# Autodesk Inventor assembly: Channel+Roller
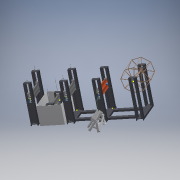
[picture p0: Inventor's stored thumbnail of the model, 180x180]
Saved by Autodesk Inventor 2019 (Build 230136000, 136)
## iProperties
Created: 2019-05-29
Part Number: Channel+Roller
Document SubType Name: Assembly
Designer: Satwik Pandey
Author: Satwik Pandey
## Documents named in this file (92)
- C:\Users\Satwik Pandey\Desktop\RuTAG Project\New folder\Channel+Roller.iam
- C:\Users\Satwik Pandey\Desktop\RuTAG Project\New folder\Channel1.ipt
- C:\Users\Satwik Pandey\Desktop\RuTAG Project\New folder\Channel2.ipt
- C:\Users\Satwik Pandey\Desktop\RuTAG Project\New folder\Extension.ipt
- C:\Users\Satwik Pandey\Desktop\RuTAG Project\New folder\Pillow Bearing inventor.ipt
- C:\Users\Satwik Pandey\Desktop\RuTAG Project\New folder\project rolller 1 part.ipt
- C:\Users\Satwik Pandey\Desktop\RuTAG Project\New folder\project rolller 1 part2.ipt
- C:\Users\Satwik Pandey\Desktop\RuTAG Project\New folder\project handle part(1).ipt
- C:\Users\Satwik Pandey\Desktop\RuTAG Project\New folder\Channel1_MIR.ipt
- C:\Users\Satwik Pandey\Desktop\RuTAG Project\New folder\Extension_MIR.ipt
- C:\Users\Satwik Pandey\Desktop\RuTAG Project\New folder\Pillow Bearing inventor_MIR.ipt
- C:\Users\Satwik Pandey\Desktop\RuTAG Project\New folder\Channel2_MIR.ipt
- C:\Users\Satwik Pandey\Desktop\RuTAG Project\New folder\project rolller 1 part_CPY.ipt
- C:\Users\Satwik Pandey\Desktop\RuTAG Project\New folder\project handle part(1)_CPY.ipt
- C:\Users\Satwik Pandey\Desktop\RuTAG Project\New folder\Channel1_MIR1.ipt
- C:\Users\Satwik Pandey\Desktop\RuTAG Project\New folder\Extension_MIR1.ipt
- C:\Users\Satwik Pandey\Desktop\RuTAG Project\New folder\Pillow Bearing inventor_MIR1.ipt
- C:\Users\Satwik Pandey\Desktop\RuTAG Project\New folder\Channel2_MIR1.ipt
- C:\Users\Satwik Pandey\Desktop\RuTAG Project\New folder\Channel1_MIR_MIR.ipt
- C:\Users\Satwik Pandey\Desktop\RuTAG Project\New folder\Extension_MIR_MIR.ipt
- C:\Users\Satwik Pandey\Desktop\RuTAG Project\New folder\Pillow Bearing inventor_MIR_MIR.ipt
- C:\Users\Satwik Pandey\Desktop\RuTAG Project\New folder\Channel2_MIR_MIR.ipt
- C:\Users\Satwik Pandey\Desktop\RuTAG Project\New folder\project handle part(1)_MIR1.ipt
- C:\Users\Satwik Pandey\Desktop\RuTAG Project\New folder\project roller 2 part1.ipt
- C:\Users\Satwik Pandey\Desktop\RuTAG Project\New folder\project roller 2 part 2.ipt
- C:\Users\Satwik Pandey\Desktop\RuTAG Project\New folder\steam pipe.ipt
- C:\Users\Satwik Pandey\Desktop\RuTAG Project\New folder\Rubber pipe.ipt
- C:\Users\Satwik Pandey\Desktop\RuTAG Project\New folder\solar heater 2.ipt
- C:\Users\Satwik Pandey\Desktop\RuTAG Project\New folder\RuTAG Roller_MIR.ipt
- C:\Users\Satwik Pandey\Desktop\RuTAG Project\New folder\Channel1_MIR4.ipt
- C:\Users\Satwik Pandey\Desktop\RuTAG Project\New folder\project flange bearing part1_MIR6.ipt
- C:\Users\Satwik Pandey\Desktop\RuTAG Project\New folder\project flange bearing part2_MIR5.ipt
- C:\Users\Satwik Pandey\Desktop\RuTAG Project\New folder\Channel1_MIR3_MIR.ipt
- C:\Users\Satwik Pandey\Desktop\RuTAG Project\New folder\project flange bearing part1_MIR5_MIR.ipt
- C:\Users\Satwik Pandey\Desktop\RuTAG Project\New folder\project flange bearing part2_MIR4_MIR.ipt
- C:\Users\Satwik Pandey\Desktop\RuTAG Project\New folder\Base1.ipt
- C:\Users\Satwik Pandey\Desktop\RuTAG Project\New folder\Base1_MIR.ipt
- C:\Users\Satwik Pandey\Desktop\RuTAG Project\New folder\Base2.ipt
- C:\Users\Satwik Pandey\Desktop\RuTAG Project\New folder\Base3.ipt
- C:\Users\Satwik Pandey\Desktop\RuTAG Project\New folder\Base4.ipt
- C:\Users\Satwik Pandey\Desktop\RuTAG Project\New folder\Channel1_MIR5.ipt
- C:\Users\Satwik Pandey\Desktop\RuTAG Project\New folder\Channel1_MIR_MIR2.ipt
- C:\Users\Satwik Pandey\Desktop\RuTAG Project\New folder\Channel1_MIR1_MIR.ipt
- C:\Users\Satwik Pandey\Desktop\RuTAG Project\New folder\Channel1_MIR_MIR_MIR.ipt
- C:\Users\Satwik Pandey\Desktop\RuTAG Project\New folder\LeadScrewArrangement.iam
- C:\Users\Satwik Pandey\Desktop\RuTAG Project\New folder\Cap1.ipt
- C:\Users\Satwik Pandey\Desktop\RuTAG Project\New folder\project handle part(1)_MIR1_MIR.ipt
- C:\Users\Satwik Pandey\Desktop\RuTAG Project\New folder\project roller 2 part1_MIR.ipt
- C:\Users\Satwik Pandey\Desktop\RuTAG Project\New folder\project roller 2 part 2_MIR.ipt
- C:\Users\Satwik Pandey\Desktop\RuTAG Project\New folder\Rubber pipe - Cap.ipt
- C:\Users\Satwik Pandey\Desktop\RuTAG Project\New folder\project flange bearing part2.ipt
- C:\Users\Satwik Pandey\Desktop\RuTAG Project\New folder\project flange bearing part1_MIR7.ipt
- C:\Users\Satwik Pandey\Desktop\RuTAG Project\New folder\project flange bearing part2_MIR6.ipt
- C:\Users\Satwik Pandey\Desktop\RuTAG Project\New folder\project flange bearing part1_MIR7_MIR.ipt
- C:\Users\Satwik Pandey\Desktop\RuTAG Project\New folder\Rubber pipe2.ipt
- C:\Users\Satwik Pandey\Desktop\RuTAG Project\New folder\Rubber pipe turn.ipt
- C:\Users\Satwik Pandey\Desktop\RuTAG Project\New folder\project flange bearing part2_MIR5_MIR.ipt
- C:\Users\Satwik Pandey\Desktop\RuTAG Project\New folder\Paste Container.ipt
- C:\Users\Satwik Pandey\Desktop\RuTAG Project\New folder\Extension_MIR3.ipt
- C:\Users\Satwik Pandey\Desktop\RuTAG Project\New folder\Pillow Bearing inventor_MIR3.ipt
- C:\Users\Satwik Pandey\Desktop\RuTAG Project\New folder\Channel2_MIR3.ipt
- C:\Users\Satwik Pandey\Desktop\RuTAG Project\New folder\Channel1_MIR6.ipt
- C:\Users\Satwik Pandey\Desktop\RuTAG Project\New folder\project rolller 1 part_MIR.ipt
- C:\Users\Satwik Pandey\Desktop\RuTAG Project\New folder\project handle part(1)_MIR2.ipt
- C:\Users\Satwik Pandey\Desktop\RuTAG Project\New folder\Extension_MIR_MIR2.ipt
- C:\Users\Satwik Pandey\Desktop\RuTAG Project\New folder\Pillow Bearing inventor_MIR_MIR2.ipt
- C:\Users\Satwik Pandey\Desktop\RuTAG Project\New folder\Channel2_MIR_MIR2.ipt
- C:\Users\Satwik Pandey\Desktop\RuTAG Project\New folder\Channel1_MIR_MIR3.ipt
- C:\Users\Satwik Pandey\Desktop\RuTAG Project\New folder\project rolller 1 part_CPY_MIR.ipt
- C:\Users\Satwik Pandey\Desktop\RuTAG Project\New folder\project handle part(1)_CPY_MIR2.ipt
- C:\Users\Satwik Pandey\Desktop\RuTAG Project\New folder\Base1_MIR1.ipt
- C:\Users\Satwik Pandey\Desktop\RuTAG Project\New folder\Channel1_MIR5_MIR.ipt
- C:\Users\Satwik Pandey\Desktop\RuTAG Project\New folder\Channel1_MIR_MIR2_MIR.ipt
- C:\Users\Satwik Pandey\Desktop\RuTAG Project\New folder\LeadScrewArrangement_MIR.iam
- C:\Users\Satwik Pandey\Desktop\RuTAG Project\New folder\Cap1_MIR1.ipt
- C:\Users\Satwik Pandey\Desktop\RuTAG Project\New folder\project flange bearing part2_MIR7.ipt
- C:\Users\Satwik Pandey\Desktop\RuTAG Project\New folder\project rolller 1 part2_MIR1.ipt
- C:\Users\Satwik Pandey\Desktop\RuTAG Project\New folder\Channel2_MIR4.ipt
- C:\Users\Satwik Pandey\Desktop\RuTAG Project\New folder\Channel1_MIR7.ipt
- C:\Users\Satwik Pandey\Desktop\RuTAG Project\New folder\Channel2_MIR_MIR3.ipt
- C:\Users\Satwik Pandey\Desktop\RuTAG Project\New folder\Channel1_MIR_MIR4.ipt
- C:\Users\Satwik Pandey\Desktop\RuTAG Project\New folder\Base1_MIR2.ipt
- C:\Users\Satwik Pandey\Desktop\RuTAG Project\New folder\Channel1_MIR5_MIR1.ipt
- C:\Users\Satwik Pandey\Desktop\RuTAG Project\New folder\Channel1_MIR_MIR2_MIR1.ipt
- C:\Users\Satwik Pandey\Desktop\RuTAG Project\New folder\project handle part.ipt
- C:\Users\Satwik Pandey\Desktop\RuTAG Project\New folder\Extension_MIR4.ipt
- C:\Users\Satwik Pandey\Desktop\RuTAG Project\New folder\Pillow Bearing inventor_MIR4.ipt
- C:\Users\Satwik Pandey\Desktop\RuTAG Project\New folder\LeadScrewArrangement_MIR1.iam
- C:\Users\Satwik Pandey\Desktop\RuTAG Project\New folder\project handle part_MIR.ipt
- C:\Users\Satwik Pandey\Desktop\RuTAG Project\New folder\project flange bearing part2_MIR8.ipt
- C:\Users\Satwik Pandey\Desktop\RuTAG Project\New folder\Cap1_MIR2.ipt
- C:\Users\Satwik Pandey\Desktop\RuTAG Project\New folder\project flange bearing part1.ipt
## Components (128 placed, 91 different names)
1. Extension:1 — Angle:8, Angle:9, Mate:5, Flush:3, Flush:4
2. Pillow Bearing inventor:1 — Angle:8, Angle:9, Mate:5, Flush:3, Flush:4, Mate:20, Mate:29
3. Channel2:1 — Flush:127, Symmetry:14
4. Channel1:3 — Symmetry:11, Mate:157, Flush:129
5. project rolller 1 part:1 — Mate:19, Flush:25, Mate:28, Symmetry:1
6. project rolller 1 part2:1 — Mate:19, Flush:25, Mate:20, Flush:38, Mate:30, Flush:39, Symmetry:1
7. project handle part(1):1 — Mate:30, Flush:39
8. project handle part(1):2 — Mate:28, Flush:38, Mate:29
9. Extension_MIR:1 — Flush:40, Flush:41, Mate:31, Angle:18, Angle:19
10. Pillow Bearing inventor_MIR:1 — Flush:40, Flush:41, Mate:31, Angle:18, Angle:19
11. Channel2_MIR:1
12. Channel1_MIR:3 — Symmetry:11, Angle:62, Flush:131, Flush:174
13. project rolller 1 part_CPY:1 — Mate:42, Mate:43, Flush:54, Mate:175
14. project handle part(1)_CPY:1 — Mate:45, Flush:55
15. project handle part(1)_CPY:2 — Mate:42, Flush:56, Mate:177
16. project rolller 1 part2:2 — Mate:43, Flush:54, Mate:45, Flush:55, Flush:56
17. Extension_MIR1:1 — Flush:60, Flush:61, Mate:50, Angle:32, Angle:33
18. Pillow Bearing inventor_MIR1:1 — Flush:60, Flush:61, Mate:50, Angle:32, Angle:33
19. Channel2_MIR1:1 — Flush:128, Symmetry:16
20. Channel1_MIR1:3 — Mate:160, Flush:138, Symmetry:17, Symmetry:18
21. Extension_MIR_MIR:1 — Angle:42, Angle:43, Mate:58, Flush:71, Flush:72
22. Pillow Bearing inventor_MIR_MIR:1 — Angle:42, Angle:43, Mate:58, Flush:71, Flush:72
23. Channel2_MIR_MIR:1
24. Channel1_MIR_MIR:3 — Symmetry:13, Mate:159, Flush:136, Symmetry:17, Flush:146
25. project handle part(1)_MIR1:1 — Mate:72
26. project handle part(1)_MIR1:2 — Flush:88, Mate:94, Mate:95, Mate:178
27. project roller 2 part1:1 — Mate:71, Flush:86, Mate:72
28. project roller 2 part 2:2 — Mate:71, Flush:86, Flush:88, Mate:93
29. steam pipe:1 — Mate:93, Mate:94, Mate:95, Mate:96, Mate:97
30. Rubber pipe:1 — Mate:96, Mate:97
31. RuTAG Roller_MIR:1 — Flush:108, Mate:106, Flush:110, Symmetry:7
32. Channel1_MIR4:1 — Mate:104, Angle:60, Mate:105, Mate:162, Flush:140, Symmetry:19
33. Channel1_MIR4:3 — Mate:102, Mate:103, Flush:139
34. project flange bearing part1_MIR6:1 — Mate:102, Mate:103, Mate:104, Angle:60, Mate:105, Flush:108, Flush:109, Mate:107
35. project flange bearing part2_MIR5:1 — Mate:106, Flush:109, Mate:107
36. Channel1_MIR3_MIR:1 — Mate:110, Angle:61, Mate:111, Mate:161
37. Channel1_MIR3_MIR:3 — Mate:112, Mate:113, Symmetry:13, Flush:133, Flush:134, Symmetry:19
38. project flange bearing part1_MIR5_MIR:1 — Mate:110, Angle:61, Mate:111, Mate:112, Mate:113, Mate:114, Flush:115
39. project flange bearing part2_MIR4_MIR:1 — Mate:114, Flush:115
40. Base1:1 — Flush:123, Mate:186, Flush:162, Mate:198
41. Base1_MIR:1 — Mate:148, Flush:120, Flush:121, Mate:149, Flush:122, Flush:145
42. Base2:1 — Flush:124, Mate:150, Flush:126, Flush:148, Flush:149, Mate:176
43. Base3:1 — Mate:148, Flush:120, Flush:121
44. Base3:2 — Mate:149, Flush:122, Flush:123
45. Base4:2 — Flush:124, Mate:150, Flush:126
46. Channel1_MIR5:1 — Symmetry:15, Angle:63, Mate:156, Flush:130
47. Channel1_MIR_MIR2:1 — Symmetry:15, Mate:154, Mate:158, Flush:132
48. Channel1_MIR1_MIR:1 — Flush:137
49. Channel1_MIR_MIR_MIR:1 — Flush:135, Flush:147, Symmetry:18
50. LeadScrewArrangement:1 [sub-assembly] — Angle:62, Mate:154
51. LeadScrewArrangement:2 [sub-assembly] — Angle:63, Mate:156
52. Cap1:1 — Mate:157, Flush:129, Flush:130
53. Cap1:2 — Mate:158, Flush:131, Flush:132
54. Cap1:3 — Mate:160, Flush:137, Flush:138
55. Cap1:4 — Mate:159, Flush:135, Flush:136
56. Cap1:5 — Mate:162, Flush:139, Flush:140
57. Cap1:6 — Mate:161, Flush:133, Flush:134
58. project handle part(1)_MIR1_MIR:1 — Mate:163, Mate:165, Mate:173
59. project handle part(1)_MIR1_MIR:2 — Mate:164
60. project roller 2 part1_MIR:1 — Mate:163
61. project roller 2 part 2_MIR:1
62. steam pipe:2 — Mate:164, Mate:165, Mate:166, Mate:167, Mate:168, Mate:169
63. Rubber pipe - Cap:1 — Mate:166, Mate:169
64. Rubber pipe - Cap:2 — Mate:167, Mate:168, Flush:151, Mate:179, Mate:181
65. project flange bearing part2:1 — Mate:173
66. project flange bearing part1_MIR7:1 — Flush:142
67. project flange bearing part2_MIR6:1 — Flush:142
68. project flange bearing part2:3 — Mate:175
69. solar heater 2:1 — Flush:145, Flush:146, Flush:147
70. Base4:3 — Flush:148, Flush:149, Mate:176
71. project flange bearing part2:4 — Mate:177
72. project flange bearing part1_MIR7_MIR:1
73. Rubber pipe2:1 — Flush:151, Mate:178, Mate:180
74. Rubber pipe turn:1 — Mate:179, Mate:180, Mate:181
75. project flange bearing part2_MIR5_MIR:1
76. Paste Container:1 — Mate:186, Flush:162, Flush:163, Symmetry:20, Mate:198, Flush:173, Symmetry:24
77. Extension_MIR3:1 — Flush:164, Flush:165, Mate:187, Angle:64, Angle:65
78. Pillow Bearing inventor_MIR3:1 — Flush:164, Flush:165, Mate:187, Angle:64, Angle:65, Mate:188
79. Channel2_MIR3:1 — Flush:168, Symmetry:22
80. Channel1_MIR6:1 — Symmetry:21, Flush:170, Mate:194
81. project rolller 1 part_MIR:1 — Mate:189
82. project handle part(1)_MIR2:1
83. project handle part(1)_MIR2:2 — Mate:188, Mate:189
84. Extension_MIR_MIR2:1 — Angle:66, Angle:67, Mate:190, Flush:166, Flush:167
85. Pillow Bearing inventor_MIR_MIR2:1 — Angle:66, Angle:67, Mate:190, Flush:166, Flush:167
86. Channel2_MIR_MIR2:1
87. Channel1_MIR_MIR3:1 — Symmetry:21, Angle:68, Flush:172
88. project rolller 1 part_CPY_MIR:1 — Mate:191, Mate:196, Mate:221
89. project handle part(1)_CPY_MIR2:1
90. project handle part(1)_CPY_MIR2:2 — Mate:191, Mate:197, Mate:219
91. Base1_MIR1:1
92. Channel1_MIR5_MIR:1 — Symmetry:23, Mate:193, Angle:69, Flush:169
93. Channel1_MIR_MIR2_MIR:1 — Symmetry:23, Mate:192, Flush:171, Mate:195
94. LeadScrewArrangement_MIR:1 [sub-assembly] — Mate:192, Angle:68, Angle:70, Mate:220
95. LeadScrewArrangement_MIR:2 [sub-assembly] — Mate:193, Angle:69, Angle:71, Mate:222
96. Cap1_MIR1:1 — Flush:169, Flush:170, Mate:194
97. Cap1_MIR1:2 — Flush:171, Flush:172, Mate:195
98. project flange bearing part2_MIR7:1 — Mate:196
99. project flange bearing part2_MIR7:2 — Mate:197
100. project rolller 1 part2_MIR1:1
101. project rolller 1 part2_MIR1:2
102. Channel2_MIR4:1 — Flush:175, Symmetry:27, Mate:199
103. Channel1_MIR7:1 — Symmetry:26, Mate:200, Mate:202, Mate:203, Flush:180, Flush:182
104. Channel2_MIR_MIR3:1
105. Channel1_MIR_MIR4:1 — Symmetry:26, Flush:176, Symmetry:29
106. Base1_MIR2:1
107. Channel1_MIR5_MIR1:1 — Symmetry:28, Flush:178, Mate:208, Flush:181
108. Channel1_MIR_MIR2_MIR1:1 — Symmetry:28
109. Extension:2 — Mate:199, Mate:200, Mate:201, Flush:177
110. Pillow Bearing inventor:2 — Mate:201, Flush:177, Mate:204, Mate:205
111. LeadScrewArrangement:3 [sub-assembly] — Flush:178, Mate:202, Mate:203, Mate:206, Flush:179
112. project handle part:1 — Mate:204, Mate:205, Mate:213, Mate:214
113. project handle part:2 — Mate:207, Mate:216, Mate:218
114. project flange bearing part2:5 — Mate:206, Flush:179, Mate:207
115. project rolller 1 part:3 — Mate:215, Flush:184
116. project rolller 1 part2:3 — Mate:213, Mate:214, Mate:215, Flush:184
117. Cap1:7 — Mate:208, Flush:181, Flush:182
118. Extension_MIR4:1 — Flush:183, Mate:209
119. Pillow Bearing inventor_MIR4:1 — Flush:183, Mate:209, Mate:210, Mate:211
120. LeadScrewArrangement_MIR1:1 [sub-assembly]
121. project handle part_MIR:1 — Mate:210, Mate:211
122. project handle part_MIR:2 — Mate:212
123. project flange bearing part2_MIR8:1 — Mate:212
124. Cap1_MIR2:1
125. project rolller 1 part:4 — Mate:217, Flush:185
126. project rolller 1 part2:4 — Mate:216, Mate:217, Mate:218, Flush:185
127. project flange bearing part1:1 — Mate:219, Angle:70, Mate:220
128. project flange bearing part1:2 — Mate:221, Angle:71, Mate:222
## Relationships (204: Mate 93, Flush 71, Angle 20, Symmetry 20)
- Angle:8 (0 deg): Extension:1 ↔ Pillow Bearing inventor:1
- Angle:9 (0 deg): Extension:1 ↔ Pillow Bearing inventor:1
- Mate:5: Extension:1 ↔ Pillow Bearing inventor:1
- Flush:3 (5 mm): Extension:1 ↔ Pillow Bearing inventor:1
- Flush:4 (-3.8 mm): Extension:1 ↔ Pillow Bearing inventor:1
- Mate:19: project rolller 1 part:1 ↔ project rolller 1 part2:1
- Flush:25: project rolller 1 part:1 ↔ project rolller 1 part2:1
- Mate:20: Pillow Bearing inventor:1 ↔ project rolller 1 part2:1
- Mate:28: project rolller 1 part:1 ↔ project handle part(1):2
- Flush:38: project rolller 1 part2:1 ↔ project handle part(1):2
- Mate:29: Pillow Bearing inventor:1 ↔ project handle part(1):2
- Mate:30: project rolller 1 part2:1 ↔ project handle part(1):1
- Flush:39: project rolller 1 part2:1 ↔ project handle part(1):1
- Symmetry:1: project rolller 1 part:1 ↔ project rolller 1 part2:1
- Flush:40 (-3.8 mm): Extension_MIR:1 ↔ Pillow Bearing inventor_MIR:1
- Flush:41 (5 mm): Extension_MIR:1 ↔ Pillow Bearing inventor_MIR:1
- Mate:31: Extension_MIR:1 ↔ Pillow Bearing inventor_MIR:1
- Angle:18 (0 deg): Extension_MIR:1 ↔ Pillow Bearing inventor_MIR:1
- Angle:19 (0 deg): Extension_MIR:1 ↔ Pillow Bearing inventor_MIR:1
- Mate:42: project rolller 1 part_CPY:1 ↔ project handle part(1)_CPY:2
- Mate:43: project rolller 1 part_CPY:1 ↔ project rolller 1 part2:2
- Flush:54: project rolller 1 part_CPY:1 ↔ project rolller 1 part2:2
- Mate:45: project handle part(1)_CPY:1 ↔ project rolller 1 part2:2
- Flush:55: project handle part(1)_CPY:1 ↔ project rolller 1 part2:2
- Flush:56: project handle part(1)_CPY:2 ↔ project rolller 1 part2:2
- Flush:60 (-3.8 mm): Extension_MIR1:1 ↔ Pillow Bearing inventor_MIR1:1
- Flush:61 (5 mm): Extension_MIR1:1 ↔ Pillow Bearing inventor_MIR1:1
- Mate:50: Extension_MIR1:1 ↔ Pillow Bearing inventor_MIR1:1
- Angle:32 (0 deg): Extension_MIR1:1 ↔ Pillow Bearing inventor_MIR1:1
- Angle:33 (0 deg): Extension_MIR1:1 ↔ Pillow Bearing inventor_MIR1:1
- Angle:42 (0 deg): Extension_MIR_MIR:1 ↔ Pillow Bearing inventor_MIR_MIR:1
- Angle:43 (0 deg): Extension_MIR_MIR:1 ↔ Pillow Bearing inventor_MIR_MIR:1
- Mate:58: Extension_MIR_MIR:1 ↔ Pillow Bearing inventor_MIR_MIR:1
- Flush:71 (5 mm): Extension_MIR_MIR:1 ↔ Pillow Bearing inventor_MIR_MIR:1
- Flush:72 (-3.8 mm): Extension_MIR_MIR:1 ↔ Pillow Bearing inventor_MIR_MIR:1
- Mate:71: project roller 2 part1:1 ↔ project roller 2 part 2:2
- Flush:86: project roller 2 part1:1 ↔ project roller 2 part 2:2
- Mate:72: project handle part(1)_MIR1:1 ↔ project roller 2 part1:1
- Flush:88: project handle part(1)_MIR1:2 ↔ project roller 2 part 2:2
- Mate:93: project roller 2 part 2:2 ↔ steam pipe:1
- Mate:94: project handle part(1)_MIR1:2 ↔ steam pipe:1
- Mate:95: project handle part(1)_MIR1:2 ↔ steam pipe:1
- Mate:96: steam pipe:1 ↔ Rubber pipe:1
- Mate:97: steam pipe:1 ↔ Rubber pipe:1
- Mate:102 (27.4 mm): Channel1_MIR4:3 ↔ project flange bearing part1_MIR6:1
- Mate:103: Channel1_MIR4:3 ↔ project flange bearing part1_MIR6:1
- Mate:104 (27.4 mm): Channel1_MIR4:1 ↔ project flange bearing part1_MIR6:1
- Angle:60 (0 deg): Channel1_MIR4:1 ↔ project flange bearing part1_MIR6:1
- Mate:105: Channel1_MIR4:1 ↔ project flange bearing part1_MIR6:1
- Flush:108 (-45 mm): RuTAG Roller_MIR:1 ↔ project flange bearing part1_MIR6:1
- Mate:106: RuTAG Roller_MIR:1 ↔ project flange bearing part2_MIR5:1
- Flush:109: project flange bearing part1_MIR6:1 ↔ project flange bearing part2_MIR5:1
- Mate:107: project flange bearing part1_MIR6:1 ↔ project flange bearing part2_MIR5:1
- Flush:110: RuTAG Roller_MIR:1
- Symmetry:7: RuTAG Roller_MIR:1
- Mate:110: Channel1_MIR3_MIR:1 ↔ project flange bearing part1_MIR5_MIR:1
- Angle:61 (0 deg): Channel1_MIR3_MIR:1 ↔ project flange bearing part1_MIR5_MIR:1
- Mate:111 (27.4 mm): Channel1_MIR3_MIR:1 ↔ project flange bearing part1_MIR5_MIR:1
- Mate:112: Channel1_MIR3_MIR:3 ↔ project flange bearing part1_MIR5_MIR:1
- Mate:113 (27.4 mm): Channel1_MIR3_MIR:3 ↔ project flange bearing part1_MIR5_MIR:1
- Mate:114: project flange bearing part1_MIR5_MIR:1 ↔ project flange bearing part2_MIR4_MIR:1
- Flush:115: project flange bearing part1_MIR5_MIR:1 ↔ project flange bearing part2_MIR4_MIR:1
- Symmetry:11: Channel1:3 ↔ Channel1_MIR:3
- Symmetry:13: Channel1_MIR_MIR:3 ↔ Channel1_MIR3_MIR:3
- Mate:148: Base1_MIR:1 ↔ Base3:1
- Flush:120: Base1_MIR:1 ↔ Base3:1
- Flush:121 (150 mm): Base1_MIR:1 ↔ Base3:1
- Mate:149: Base1_MIR:1 ↔ Base3:2
- Flush:122: Base1_MIR:1 ↔ Base3:2
- Flush:123 (-150 mm): Base1:1 ↔ Base3:2
- Flush:124: Base2:1 ↔ Base4:2
- Mate:150: Base2:1 ↔ Base4:2
- Flush:126 (-150 mm): Base2:1 ↔ Base4:2
- Flush:127: Channel2:1
- Symmetry:14: Channel2:1
- Symmetry:15: Channel1_MIR5:1 ↔ Channel1_MIR_MIR2:1
- Flush:128: Channel2_MIR1:1
- Symmetry:16: Channel2_MIR1:1
- Angle:62 (0 deg): Channel1_MIR:3 ↔ LeadScrewArrangement:1
- Mate:154: Channel1_MIR_MIR2:1 ↔ LeadScrewArrangement:1
- Angle:63 (180 deg): Channel1_MIR5:1 ↔ LeadScrewArrangement:2
- Mate:156: Channel1_MIR5:1 ↔ LeadScrewArrangement:2
- Mate:157: Channel1:3 ↔ Cap1:1
- Flush:129: Channel1:3 ↔ Cap1:1
- Flush:130: Channel1_MIR5:1 ↔ Cap1:1
- Mate:158: Channel1_MIR_MIR2:1 ↔ Cap1:2
- Flush:131: Channel1_MIR:3 ↔ Cap1:2
- Flush:132: Channel1_MIR_MIR2:1 ↔ Cap1:2
- Mate:159: Channel1_MIR_MIR:3 ↔ Cap1:4
- Mate:160: Channel1_MIR1:3 ↔ Cap1:3
- Mate:161: Channel1_MIR3_MIR:1 ↔ Cap1:6
- Mate:162: Channel1_MIR4:1 ↔ Cap1:5
- Flush:133: Channel1_MIR3_MIR:3 ↔ Cap1:6
- Flush:134: Channel1_MIR3_MIR:3 ↔ Cap1:6
- Flush:135: Channel1_MIR_MIR_MIR:1 ↔ Cap1:4
- Flush:136: Channel1_MIR_MIR:3 ↔ Cap1:4
- Flush:137: Channel1_MIR1_MIR:1 ↔ Cap1:3
- Flush:138: Channel1_MIR1:3 ↔ Cap1:3
- Flush:139: Channel1_MIR4:3 ↔ Cap1:5
- Flush:140: Channel1_MIR4:1 ↔ Cap1:5
- Mate:163: project handle part(1)_MIR1_MIR:1 ↔ project roller 2 part1_MIR:1
- Mate:164: project handle part(1)_MIR1_MIR:2 ↔ steam pipe:2
- Mate:165 (5 mm): project handle part(1)_MIR1_MIR:1 ↔ steam pipe:2
- Mate:166: steam pipe:2 ↔ Rubber pipe - Cap:1
- Mate:167: steam pipe:2 ↔ Rubber pipe - Cap:2
- Mate:168: steam pipe:2 ↔ Rubber pipe - Cap:2
- Mate:169 (-10 mm): steam pipe:2 ↔ Rubber pipe - Cap:1
- Mate:173: project handle part(1)_MIR1_MIR:1 ↔ project flange bearing part2:1
- Symmetry:17: Channel1_MIR1:3 ↔ Channel1_MIR_MIR:3
- Flush:142: project flange bearing part1_MIR7:1 ↔ project flange bearing part2_MIR6:1
- Mate:175: project rolller 1 part_CPY:1 ↔ project flange bearing part2:3
- Flush:145: Base1_MIR:1 ↔ solar heater 2:1
- Flush:146 (600 mm): Channel1_MIR_MIR:3 ↔ solar heater 2:1
- Flush:147 (-120 mm): Channel1_MIR_MIR_MIR:1 ↔ solar heater 2:1
- Flush:148: Base2:1 ↔ Base4:3
- Flush:149 (150 mm): Base2:1 ↔ Base4:3
- Mate:176: Base2:1 ↔ Base4:3
- Mate:177: project handle part(1)_CPY:2 ↔ project flange bearing part2:4
- Symmetry:18: Channel1_MIR1:3 ↔ Channel1_MIR_MIR_MIR:1
- Flush:151: Rubber pipe - Cap:2 ↔ Rubber pipe2:1
- Mate:178: project handle part(1)_MIR1:2 ↔ Rubber pipe2:1
- Mate:179: Rubber pipe - Cap:2 ↔ Rubber pipe turn:1
- Mate:180: Rubber pipe2:1 ↔ Rubber pipe turn:1
- Mate:181: Rubber pipe - Cap:2 ↔ Rubber pipe turn:1
- Symmetry:19: Channel1_MIR4:1 ↔ Channel1_MIR3_MIR:3
- Mate:186 (50 mm): Base1:1 ↔ Paste Container:1
- Flush:162: Base1:1 ↔ Paste Container:1
- Flush:163: Paste Container:1
- Symmetry:20: Paste Container:1
- Flush:164 (-3.8 mm): Extension_MIR3:1 ↔ Pillow Bearing inventor_MIR3:1
- Flush:165 (5 mm): Extension_MIR3:1 ↔ Pillow Bearing inventor_MIR3:1
- Mate:187: Extension_MIR3:1 ↔ Pillow Bearing inventor_MIR3:1
- Angle:64 (0 deg): Extension_MIR3:1 ↔ Pillow Bearing inventor_MIR3:1
- Angle:65 (0 deg): Extension_MIR3:1 ↔ Pillow Bearing inventor_MIR3:1
- Mate:188: Pillow Bearing inventor_MIR3:1 ↔ project handle part(1)_MIR2:2
- Mate:189: project rolller 1 part_MIR:1 ↔ project handle part(1)_MIR2:2
- Angle:66 (0 deg): Extension_MIR_MIR2:1 ↔ Pillow Bearing inventor_MIR_MIR2:1
- Angle:67 (0 deg): Extension_MIR_MIR2:1 ↔ Pillow Bearing inventor_MIR_MIR2:1
- Mate:190: Extension_MIR_MIR2:1 ↔ Pillow Bearing inventor_MIR_MIR2:1
- Flush:166 (5 mm): Extension_MIR_MIR2:1 ↔ Pillow Bearing inventor_MIR_MIR2:1
- Flush:167 (-3.8 mm): Extension_MIR_MIR2:1 ↔ Pillow Bearing inventor_MIR_MIR2:1
- Mate:191: project rolller 1 part_CPY_MIR:1 ↔ project handle part(1)_CPY_MIR2:2
- Symmetry:21: Channel1_MIR6:1 ↔ Channel1_MIR_MIR3:1
- Flush:168: Channel2_MIR3:1
- Symmetry:22: Channel2_MIR3:1
- Symmetry:23: Channel1_MIR5_MIR:1 ↔ Channel1_MIR_MIR2_MIR:1
- Mate:192: Channel1_MIR_MIR2_MIR:1 ↔ LeadScrewArrangement_MIR:1
- Angle:68 (0 deg): Channel1_MIR_MIR3:1 ↔ LeadScrewArrangement_MIR:1
- Mate:193: Channel1_MIR5_MIR:1 ↔ LeadScrewArrangement_MIR:2
- Angle:69 (180 deg): Channel1_MIR5_MIR:1 ↔ LeadScrewArrangement_MIR:2
- Flush:169: Channel1_MIR5_MIR:1 ↔ Cap1_MIR1:1
- Flush:170: Channel1_MIR6:1 ↔ Cap1_MIR1:1
- Mate:194: Channel1_MIR6:1 ↔ Cap1_MIR1:1
- Flush:171: Channel1_MIR_MIR2_MIR:1 ↔ Cap1_MIR1:2
- Flush:172: Channel1_MIR_MIR3:1 ↔ Cap1_MIR1:2
- Mate:195: Channel1_MIR_MIR2_MIR:1 ↔ Cap1_MIR1:2
- Mate:196: project rolller 1 part_CPY_MIR:1 ↔ project flange bearing part2_MIR7:1
- Mate:197: project handle part(1)_CPY_MIR2:2 ↔ project flange bearing part2_MIR7:2
- Mate:198: Base1:1 ↔ Paste Container:1
- Flush:173: Paste Container:1
- Symmetry:24: Paste Container:1
- Flush:174 (-97 mm): Channel1_MIR:3
- Symmetry:25
- Symmetry:26: Channel1_MIR7:1 ↔ Channel1_MIR_MIR4:1
- Flush:175: Channel2_MIR4:1
- Symmetry:27: Channel2_MIR4:1
- Symmetry:28: Channel1_MIR5_MIR1:1 ↔ Channel1_MIR_MIR2_MIR1:1
- Flush:176 (-97 mm): Channel1_MIR_MIR4:1
- Mate:199: Channel2_MIR4:1 ↔ Extension:2
- Mate:200: Channel1_MIR7:1 ↔ Extension:2
- Mate:201: Extension:2 ↔ Pillow Bearing inventor:2
- Flush:177: Extension:2 ↔ Pillow Bearing inventor:2
- Flush:178 (20 mm): Channel1_MIR5_MIR1:1 ↔ LeadScrewArrangement:3
- Mate:202 (18 mm): Channel1_MIR7:1 ↔ LeadScrewArrangement:3
- Mate:203: Channel1_MIR7:1 ↔ LeadScrewArrangement:3
- Mate:204: Pillow Bearing inventor:2 ↔ project handle part:1
- Mate:205: Pillow Bearing inventor:2 ↔ project handle part:1
- Mate:206: LeadScrewArrangement:3 ↔ project flange bearing part2:5
- Flush:179: LeadScrewArrangement:3 ↔ project flange bearing part2:5
- Mate:207: project handle part:2 ↔ project flange bearing part2:5
- Flush:180: Channel1_MIR7:1
- Symmetry:29: Channel1_MIR_MIR4:1
- Mate:208: Channel1_MIR5_MIR1:1 ↔ Cap1:7
- Flush:181: Channel1_MIR5_MIR1:1 ↔ Cap1:7
- Flush:182: Channel1_MIR7:1 ↔ Cap1:7
- Flush:183: Extension_MIR4:1 ↔ Pillow Bearing inventor_MIR4:1
- Mate:209: Extension_MIR4:1 ↔ Pillow Bearing inventor_MIR4:1
- Mate:210: Pillow Bearing inventor_MIR4:1 ↔ project handle part_MIR:1
- Mate:211: Pillow Bearing inventor_MIR4:1 ↔ project handle part_MIR:1
- Mate:212: project handle part_MIR:2 ↔ project flange bearing part2_MIR8:1
- Mate:213: project handle part:1 ↔ project rolller 1 part2:3
- Mate:214: project handle part:1 ↔ project rolller 1 part2:3
- Mate:215: project rolller 1 part:3 ↔ project rolller 1 part2:3
- Flush:184: project rolller 1 part:3 ↔ project rolller 1 part2:3
- Mate:216: project handle part:2 ↔ project rolller 1 part2:4
- Mate:217: project rolller 1 part:4 ↔ project rolller 1 part2:4
- Mate:218: project handle part:2 ↔ project rolller 1 part2:4
- Flush:185: project rolller 1 part:4 ↔ project rolller 1 part2:4
- Mate:219: project handle part(1)_CPY_MIR2:2 ↔ project flange bearing part1:1
- Angle:70 (0 deg): LeadScrewArrangement_MIR:1 ↔ project flange bearing part1:1
- Mate:220: LeadScrewArrangement_MIR:1 ↔ project flange bearing part1:1
- Mate:221: project rolller 1 part_CPY_MIR:1 ↔ project flange bearing part1:2
- Angle:71 (0 deg): LeadScrewArrangement_MIR:2 ↔ project flange bearing part1:2
- Mate:222: LeadScrewArrangement_MIR:2 ↔ project flange bearing part1:2
